# Autodesk Inventor assembly: TOTEM_Slider_X
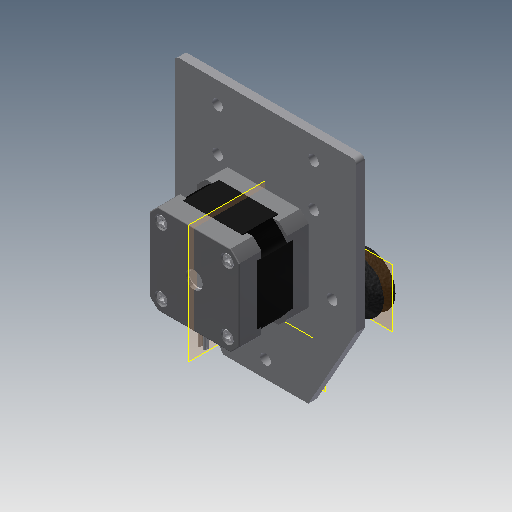
[picture p0: Inventor's stored thumbnail of the model, 512x512]
Saved by Autodesk Inventor 2019.4 (Build 234330000, 330)
## iProperties
Created: 2021-10-12
Part Number: TOTEM_Slider_X
Document SubType Name: Assembly
Designer: diederichbenedict
Author: diederichbenedict
## Documents named in this file (4)
- C:\Users\diederichbenedict\Dropbox\Dokumente\Promotion\PROJECTS\UC2\02_CAD\INVENTOR\uc2_v3\TOTEM_Slider_X.iam
- C:\Users\diederichbenedict\Dropbox\Dokumente\Promotion\PROJECTS\UC2\02_CAD\INVENTOR\uc2_v3\TOTEM_Base_Slide_x_20mmrod.ipt
- C:\Users\diederichbenedict\Dropbox\Dokumente\Promotion\PROJECTS\UC2\02_CAD\INVENTOR\uc2_v3\00_NEMA17.ipt
- C:\Users\diederichbenedict\Dropbox\Dokumente\Promotion\PROJECTS\UC2\02_CAD\INVENTOR\uc2_v3\Neje_Rolls.ipt
## Components (5 placed, 3 different names)
1. TOTEM_Base_Slide_x_20mmrod:1 — Insert:1, Angle:1, Insert:2, Insert:3, Insert:4
2. 00_NEMA17:1 — Insert:1, Angle:1
3. Neje_Rolls:1 — Insert:3
4. Neje_Rolls:2 — Insert:2
5. Neje_Rolls:3 — Insert:4
## Relationships (5: Insert 4, Angle 1)
- Insert:1: TOTEM_Base_Slide_x_20mmrod:1 ↔ 00_NEMA17:1
- Angle:1 (180 deg): TOTEM_Base_Slide_x_20mmrod:1 ↔ 00_NEMA17:1
- Insert:2 (5 mm): TOTEM_Base_Slide_x_20mmrod:1 ↔ Neje_Rolls:2
- Insert:3 (5 mm): TOTEM_Base_Slide_x_20mmrod:1 ↔ Neje_Rolls:1
- Insert:4 (5 mm): TOTEM_Base_Slide_x_20mmrod:1 ↔ Neje_Rolls:3
